# Autodesk Inventor assembly: computer assembly
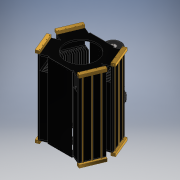
[picture p0: Inventor's stored thumbnail of the model, 180x180]
Saved by Autodesk Inventor 2018 (Build 220112000, 112)
## iProperties
Created: 2018-06-04
Part Number: computer assembly
Document SubType Name: Assembly
Designer: John Viljoen
Author: John Viljoen
## Documents named in this file (10)
- C:\Users\John Viljoen\Documents\Inventor\computer project\computer assembly.iam
- C:\Users\John Viljoen\Documents\Inventor\computer project\baseplate.ipt
- C:\Users\John Viljoen\Documents\Inventor\computer project\coverplate.ipt
- C:\Users\John Viljoen\Documents\Inventor\computer project\topplate.ipt
- C:\Users\John Viljoen\Documents\Inventor\computer project\heat sink.ipt
- C:\Users\John Viljoen\Documents\Inventor\computer project\manifold.ipt
- C:\Users\John Viljoen\Documents\Inventor\computer project\manifold mirror.ipt
- C:\Users\John Viljoen\Documents\Inventor\computer project\sideplate.ipt
- C:\Users\John Viljoen\Documents\Inventor\computer project\grabcad reservoir pump combo.iam
- C:\Users\John Viljoen\Documents\Inventor\computer project\coverplate pipe.ipt
## Components (33 placed, 9 different names)
1. baseplate:1 — Mate:9, Flush:5, Flush:6, Mate:11, Mate:13, Mate:15, Mate:17, Mate:20, Flush:12, Mate:24, Flush:14, Mate:30, Flush:17, Mate:32, Flush:18, Flush:23
2. coverplate:1 — Mate:7, Mate:8, Flush:4, Mate:16, Flush:10, Mate:27, Mate:33, Mate:43, Mate:45, Mate:47
3. coverplate:2 — Mate:1, Mate:2, Flush:1, Mate:12, Flush:8, Mate:19, Mate:21, Mate:55, Mate:57, Mate:59
4. coverplate:3 — Mate:5, Mate:6, Flush:3, Mate:9, Flush:5, Flush:6, Mate:14, Flush:9, Mate:23, Mate:25, Mate:37, Mate:39, Mate:41
5. coverplate:4 — Mate:3, Mate:4, Flush:2, Mate:10, Flush:7, Mate:29, Mate:31, Mate:49, Mate:51, Mate:53
6. topplate:1 — Mate:1, Mate:2, Flush:1, Mate:3, Mate:4, Flush:2, Mate:5, Mate:6, Flush:3, Mate:7, Mate:8, Flush:4, Mate:18, Flush:11, Mate:22, Flush:13, Mate:26, Flush:15, Mate:28, Flush:16, Mate:34, Flush:19, Flush:20, Mate:35, Flush:21, Flush:22
7. heat sink:1 — Mate:12, Flush:8, Mate:13
8. heat sink:2 — Mate:14, Flush:9, Mate:15
9. heat sink:3 — Mate:16, Flush:10, Mate:17
10. heat sink:4 — Mate:10, Mate:11, Flush:7
11. manifold:1 — Mate:18, Flush:11, Mate:19, Mate:56, Mate:58, Mate:60
12. manifold:2 — Mate:20, Flush:12, Mate:21
13. manifold:3 — Mate:24, Flush:14, Mate:25
14. manifold:4 — Mate:22, Flush:13, Mate:23, Mate:38, Mate:40, Mate:42
15. manifold mirror:1 — Mate:26, Flush:15, Mate:27, Mate:44, Mate:46, Mate:48
16. manifold mirror:2 — Mate:28, Flush:16, Mate:29, Mate:50, Mate:52, Mate:54
17. manifold mirror:3 — Mate:30, Flush:17, Mate:31
18. manifold mirror:4 — Mate:32, Flush:18, Mate:33
19. sideplate:1 — Mate:34, Flush:19, Flush:20
20. sideplate:2 — Mate:35, Flush:21, Flush:22, Mate:36, Flush:24
21. grabcad reservoir pump combo:1 [sub-assembly] — Mate:36, Flush:23, Flush:24
22. coverplate pipe:1 — Mate:37, Mate:38
23. coverplate pipe:2 — Mate:39, Mate:40
24. coverplate pipe:3 — Mate:41, Mate:42
25. coverplate pipe:4 — Mate:43, Mate:44
26. coverplate pipe:5 — Mate:45, Mate:46
27. coverplate pipe:6 — Mate:47, Mate:48
28. coverplate pipe:7 — Mate:49, Mate:50
29. coverplate pipe:8 — Mate:51, Mate:52
30. coverplate pipe:9 — Mate:53, Mate:54
31. coverplate pipe:10 — Mate:55, Mate:56
32. coverplate pipe:11 — Mate:57, Mate:58
33. coverplate pipe:12 — Mate:59, Mate:60
## Relationships (84: Mate 60, Flush 24)
- Mate:1: coverplate:2 ↔ topplate:1
- Mate:2: coverplate:2 ↔ topplate:1
- Flush:1: coverplate:2 ↔ topplate:1
- Mate:3: coverplate:4 ↔ topplate:1
- Mate:4: coverplate:4 ↔ topplate:1
- Flush:2: coverplate:4 ↔ topplate:1
- Mate:5: coverplate:3 ↔ topplate:1
- Mate:6: coverplate:3 ↔ topplate:1
- Flush:3: coverplate:3 ↔ topplate:1
- Mate:7: coverplate:1 ↔ topplate:1
- Mate:8: coverplate:1 ↔ topplate:1
- Flush:4: coverplate:1 ↔ topplate:1
- Mate:9: baseplate:1 ↔ coverplate:3
- Flush:5: baseplate:1 ↔ coverplate:3
- Flush:6: baseplate:1 ↔ coverplate:3
- Mate:10: coverplate:4 ↔ heat sink:4
- Mate:11: baseplate:1 ↔ heat sink:4
- Flush:7: coverplate:4 ↔ heat sink:4
- Mate:12: coverplate:2 ↔ heat sink:1
- Flush:8: coverplate:2 ↔ heat sink:1
- Mate:13: baseplate:1 ↔ heat sink:1
- Mate:14: coverplate:3 ↔ heat sink:2
- Flush:9: coverplate:3 ↔ heat sink:2
- Mate:15: baseplate:1 ↔ heat sink:2
- Mate:16: coverplate:1 ↔ heat sink:3
- Flush:10: coverplate:1 ↔ heat sink:3
- Mate:17: baseplate:1 ↔ heat sink:3
- Mate:18: topplate:1 ↔ manifold:1
- Flush:11: topplate:1 ↔ manifold:1
- Mate:19: coverplate:2 ↔ manifold:1
- Mate:20: baseplate:1 ↔ manifold:2
- Flush:12: baseplate:1 ↔ manifold:2
- Mate:21: coverplate:2 ↔ manifold:2
- Mate:22: topplate:1 ↔ manifold:4
- Flush:13: topplate:1 ↔ manifold:4
- Mate:23: coverplate:3 ↔ manifold:4
- Mate:24: baseplate:1 ↔ manifold:3
- Flush:14: baseplate:1 ↔ manifold:3
- Mate:25: coverplate:3 ↔ manifold:3
- Mate:26: topplate:1 ↔ manifold mirror:1
- Flush:15: topplate:1 ↔ manifold mirror:1
- Mate:27: coverplate:1 ↔ manifold mirror:1
- Mate:28: topplate:1 ↔ manifold mirror:2
- Flush:16: topplate:1 ↔ manifold mirror:2
- Mate:29: coverplate:4 ↔ manifold mirror:2
- Mate:30: baseplate:1 ↔ manifold mirror:3
- Flush:17: baseplate:1 ↔ manifold mirror:3
- Mate:31: coverplate:4 ↔ manifold mirror:3
- Mate:32: baseplate:1 ↔ manifold mirror:4
- Flush:18: baseplate:1 ↔ manifold mirror:4
- Mate:33: coverplate:1 ↔ manifold mirror:4
- Mate:34: topplate:1 ↔ sideplate:1
- Flush:19: topplate:1 ↔ sideplate:1
- Flush:20: topplate:1 ↔ sideplate:1
- Mate:35: topplate:1 ↔ sideplate:2
- Flush:21: topplate:1 ↔ sideplate:2
- Flush:22: topplate:1 ↔ sideplate:2
- Mate:36: sideplate:2 ↔ grabcad reservoir pump combo:1
- Flush:23 (50 mm): baseplate:1 ↔ grabcad reservoir pump combo:1
- Flush:24 (32 mm): sideplate:2 ↔ grabcad reservoir pump combo:1
- Mate:37: coverplate:3 ↔ coverplate pipe:1
- Mate:38 (-2 mm): manifold:4 ↔ coverplate pipe:1
- Mate:39: coverplate:3 ↔ coverplate pipe:2
- Mate:40 (-2 mm): manifold:4 ↔ coverplate pipe:2
- Mate:41: coverplate:3 ↔ coverplate pipe:3
- Mate:42 (-2 mm): manifold:4 ↔ coverplate pipe:3
- Mate:43: coverplate:1 ↔ coverplate pipe:4
- Mate:44 (-2 mm): manifold mirror:1 ↔ coverplate pipe:4
- Mate:45: coverplate:1 ↔ coverplate pipe:5
- Mate:46 (-2 mm): manifold mirror:1 ↔ coverplate pipe:5
- Mate:47: coverplate:1 ↔ coverplate pipe:6
- Mate:48 (-2 mm): manifold mirror:1 ↔ coverplate pipe:6
- Mate:49: coverplate:4 ↔ coverplate pipe:7
- Mate:50 (-2 mm): manifold mirror:2 ↔ coverplate pipe:7
- Mate:51: coverplate:4 ↔ coverplate pipe:8
- Mate:52 (-2 mm): manifold mirror:2 ↔ coverplate pipe:8
- Mate:53: coverplate:4 ↔ coverplate pipe:9
- Mate:54 (-2 mm): manifold mirror:2 ↔ coverplate pipe:9
- Mate:55: coverplate:2 ↔ coverplate pipe:10
- Mate:56 (-2 mm): manifold:1 ↔ coverplate pipe:10
- Mate:57: coverplate:2 ↔ coverplate pipe:11
- Mate:58 (-2 mm): manifold:1 ↔ coverplate pipe:11
- Mate:59: coverplate:2 ↔ coverplate pipe:12
- Mate:60 (-2 mm): manifold:1 ↔ coverplate pipe:12
